# Autodesk Inventor assembly: Arm Linkage
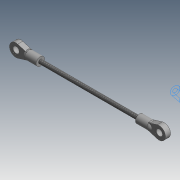
[picture p0: Inventor's stored thumbnail of the model, 180x180]
Saved by Autodesk Inventor 2014 SP1 (Build 180222100, 222)
## iProperties
Created: 2014-04-09
Part Number: Arm Linkage
Document SubType Name: Assembly
Designer: tom
Author: tom
## Documents named in this file (3)
- C:\Users\tom\Documents\GitHub\Delta_Robots\Delatabot - Small Model\Inventor\Deltabot - Small Model ver12\Arm Linkage.iam
- C:\Users\tom\Documents\GitHub\Delta_Robots\Delatabot - Small Model\Inventor\Deltabot - Small Model ver12\Body.ipt
- C:\Users\tom\Documents\GitHub\Delta_Robots\Delatabot - Small Model\Inventor\Deltabot - Small Model ver12\6-32 Rod.ipt
## Components (3 placed, 2 different names)
1. Body:1
2. 6-32 Rod:1
3. Body:2
## Relationships (3: Mate 3)
- [Mate]: 6-32 Rod:1 ↔ Body:2
- [Mate]: 6-32 Rod:1 ↔ Body:2
- [Mate]: Body:1 ↔ 6-32 Rod:1
